# Autodesk Inventor assembly: DockingHolder_CommercialNP2
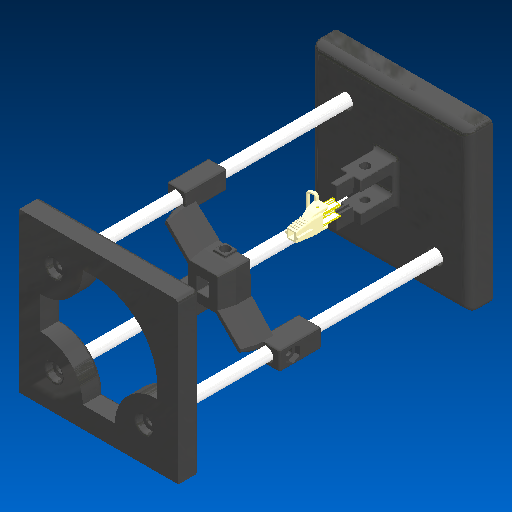
[picture p0: Inventor's stored thumbnail of the model, 512x512]
Saved by Autodesk Inventor 2025 (Build 290162000, 162)
## iProperties
Created: 2024-10-31
Part Number: DockingHolder_CommercialNP2
Document SubType Name: Assembly
Designer: AdminForWorker
Mass: 118.03 g
Surface Area: 432.107 cm^2
Volume: 117.991 cm^3
Density: 1.00033 g/cm^3
Title: NP2_DockingHolder v28
Author: AdminForWorker
## Documents named in this file (7)
- C:\Users\faricci\Coen\chronic-neuropixels\XtraModifications\Mouse_FreelyMoving\New_Mounting\NP2_mounting_bigger\NP2_DockingHolder_bigger.iam
- C:\Users\faricci\Coen\chronic-neuropixels\XtraModifications\Mouse_FreelyMoving\New_Mounting\NP2_mounting_bigger\NP2_DockingHolder_bigger.ipt
- C:\Users\faricci\Coen\chronic-neuropixels\XtraModifications\Mouse_FreelyMoving\New_Mounting\NP2_mounting_bigger\NP2_PayloadHolder v1_bigger.ipt
- C:\Users\faricci\Coen\chronic-neuropixels\XtraModifications\Mouse_FreelyMoving\New_Mounting\NP2_mounting_bigger\Bars.ipt
- C:\Users\faricci\Coen\chronic-neuropixels\XtraModifications\Mouse_FreelyMoving\New_Mounting\NP2_mounting_bigger\ConstructorHead_bigger.ipt
- C:\Users\faricci\Coen\chronic-neuropixels\XtraModifications\Mouse_FreelyMoving\New_Mounting\NP2_SingleProbeDockingWithHeadstage_FullyParameterised_fin.ipt
- C:\Users\faricci\Coen\chronic-neuropixels\XtraModifications\Mouse_FreelyMoving\New_Mounting\NP2_SingleProbeMiniaturePayload.ipt
## Components (6 placed, 6 different names)
1. Bigger_NP2_DockingHolder:1 — Slider:1
2. NP2_PayloadHolder v1:1 — Rigid:1
3. Bars:1 — Rigid:1, Rigid:2
4. Part12 — Rigid:2
5. NP2_SingleProbeDockingWithHeadstage_FullyParameterised_fin:1 — Slider:1
6. NP2_SingleProbeMiniaturePayload:1
## Relationships (3: WeldJoint 2, TranslationJoint 1)
- Rigid:1 [WeldJoint]: NP2_PayloadHolder v1:1 ↔ Bars:1
- Rigid:2 [WeldJoint]: Bars:1 ↔ Part12
- Slider:1 [TranslationJoint] (0.4 mm): Bigger_NP2_DockingHolder:1 ↔ NP2_SingleProbeDockingWithHeadstage_FullyParameterised_fin:1
